# Autodesk Inventor assembly: SloppyAssembly
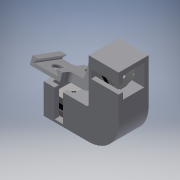
[picture p0: Inventor's stored thumbnail of the model, 180x180]
Saved by Autodesk Inventor 2017 (Build 210142000, 142)
## iProperties
Created: 2017-01-06
Part Number: SloppyAssembly
Document SubType Name: Assembly
Designer: kurti
Author: kurti
## Documents named in this file (4)
- D:\Users\kurti\Git Home\CAD\Sentry Camera\V2CAD\SloppyAssembly.iam
- D:\Users\kurti\Git Home\CAD\Sentry Camera\V2CAD\OuterFrame.ipt
- D:\Users\kurti\Git Home\CAD\Sentry Camera\cad\assets\SmallStepper.ipt
- D:\Users\kurti\Git Home\CAD\Sentry Camera\V2CAD\InnerFrameSimple.ipt
## Components (4 placed, 3 different names)
1. OuterFrame:1 — Rotational:1, Rotational:2
2. SmallStepper:1 — Rotational:1
3. SmallStepper:2 — Rotational:2, Rotational:3
4. InnerFrameSimple:1 — Rotational:3
## Relationships (3: RevoluteJoint 3)
- Rotational:1 [RevoluteJoint]: OuterFrame:1 ↔ SmallStepper:1
- Rotational:2 [RevoluteJoint]: OuterFrame:1 ↔ SmallStepper:2
- Rotational:3 [RevoluteJoint]: SmallStepper:2 ↔ InnerFrameSimple:1
